# Autodesk Inventor assembly: simp_burnisher_w100roller
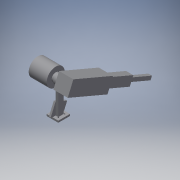
[picture p0: Inventor's stored thumbnail of the model, 180x180]
Saved by Autodesk Inventor 2019 (Build 230136000, 136)
## iProperties
Created: 2019-11-07
Part Number: simp_burnisher_w100roller
Document SubType Name: Assembly
Designer: luua
Author: luua
## Documents named in this file (3)
- C:\Users\Pengj5\OneDrive - Queensland University of Technology\Documents\bracket\metabo-burnisher-model\simp_burnisher_w100roller.iam
- C:\Users\Pengj5\OneDrive - Queensland University of Technology\Documents\bracket\metabo-burnisher-model\simp_burnisher.ipt
- C:\Users\Pengj5\OneDrive - Queensland University of Technology\Documents\bracket\metabo-burnisher-model\100mm_roller.ipt
## Components (2 placed, 2 different names)
1. simp_burnisher:1 — Mate:1, Mate:2, Flush:1, Mate:3
2. 100mm_roller:1 — Mate:1
## Relationships (4: Mate 3, Flush 1)
- Mate:1: simp_burnisher:1 ↔ 100mm_roller:1
- Mate:2: simp_burnisher:1
- Flush:1: simp_burnisher:1
- Mate:3: simp_burnisher:1
